# Autodesk Inventor assembly: Lift.03.02.00.00
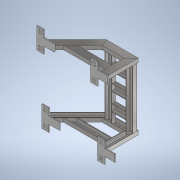
[picture p0: Inventor's stored thumbnail of the model, 180x180]
Saved by Autodesk Inventor 2021 (Build 250183000, 183)
## iProperties
_SolveAssemblyDoc: Frame Generator Solve Assembly
_Version: 15.0.0
Created: 2020-09-20
Part Number: Lift.03.02.00.00
Document SubType Name: Assembly
Designer: Kostya
Author: Kostya
## Documents named in this file (4)
- C:\Lift\Lift.03.02.00.00.iam
- C:\Lift\Lift.03.02.00.01.ipt
- C:\Lift\Lift.03.02.00.02.ipt
- C:\Lift\Lift.03.02.00.00\Frame\Frame 1600618668392.iam
## Components (6 placed, 3 different names)
1. Lift.03.02.00.01:1 — Совмещение:1
2. Lift.03.02.00.02:1
3. Frame 1600618668392:1 [sub-assembly] — Совмещение:1, Совмещение:2, Совмещение:3, Совмещение:4
4. Lift.03.02.00.01:2 — Совмещение:3
5. Lift.03.02.00.01:3 — Совмещение:4
6. Lift.03.02.00.01:4 — Совмещение:2
## Relationships (4: Mate 4)
- Совмещение:1 [Mate]: Lift.03.02.00.01:1 ↔ Frame 1600618668392:1
- Совмещение:2 [Mate]: Frame 1600618668392:1 ↔ Lift.03.02.00.01:4
- Совмещение:3 [Mate]: Frame 1600618668392:1 ↔ Lift.03.02.00.01:2
- Совмещение:4 [Mate]: Frame 1600618668392:1 ↔ Lift.03.02.00.01:3
